# Autodesk Inventor assembly: Pusher2
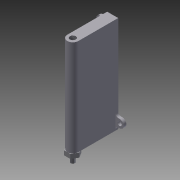
[picture p0: Inventor's stored thumbnail of the model, 180x180]
Saved by Autodesk Inventor 2011 (Build 150239000, 239)
## iProperties
Created: 2011-04-12
Part Number: Pusher2
Document SubType Name: Assembly
Designer: Rob
Author: Rob
## Documents named in this file (5)
- C:\Users\Rob\Dropbox\RockSAT-X 2011 RexSAT\capsule-launcher.design\Launcher\Pusher2.iam
- C:\Users\Rob\Dropbox\RockSAT-X 2011 RexSAT\capsule-launcher.design\Launcher\Pusher.Holder2.ipt
- C:\Users\Rob\Dropbox\RockSAT-X 2011 RexSAT\capsule-launcher.design\Launcher\Pusher.springplate.ipt
- C:\Users\Rob\Dropbox\RockSAT-X 2011 RexSAT\capsule-launcher.design\Launcher\Pusher.Bolt.ipt
- C:\Users\Rob\Dropbox\RockSAT-X 2011 RexSAT\capsule-launcher.design\Launcher\Pusher.Pushrod.ipt
## Components (6 placed, 4 different names)
1. Pusher.Holder2:1 — Flush:1, Mate:1, Flush:2, Mate:2, Flush:3, Mate:3, Mate:4, Mate:5, Mate:8
2. Pusher.springplate:2 — Flush:3, Mate:3
3. Pusher.springplate:3 — Flush:2, Mate:2
4. Pusher.springplate:4 — Flush:1, Mate:1
5. Pusher.Bolt:1 — Mate:4, Mate:5, Mate:7, Flush:4
6. Pusher.Pushrod:1 — Mate:7, Mate:8, Flush:4
## Relationships (11: Mate 7, Flush 4)
- Flush:1 (9.603 mm): Pusher.Holder2:1 ↔ Pusher.springplate:4
- Mate:1: Pusher.Holder2:1 ↔ Pusher.springplate:4
- Flush:2 (44.512 mm): Pusher.Holder2:1 ↔ Pusher.springplate:3
- Mate:2: Pusher.Holder2:1 ↔ Pusher.springplate:3
- Flush:3 (79.412 mm): Pusher.Holder2:1 ↔ Pusher.springplate:2
- Mate:3: Pusher.Holder2:1 ↔ Pusher.springplate:2
- Mate:4: Pusher.Holder2:1 ↔ Pusher.Bolt:1
- Mate:5: Pusher.Holder2:1 ↔ Pusher.Bolt:1
- Mate:7: Pusher.Bolt:1 ↔ Pusher.Pushrod:1
- Mate:8: Pusher.Holder2:1 ↔ Pusher.Pushrod:1
- Flush:4 (-10 mm): Pusher.Bolt:1 ↔ Pusher.Pushrod:1
